# Autodesk Inventor assembly: FinalAssembley
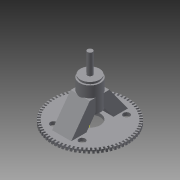
[picture p0: Inventor's stored thumbnail of the model, 180x180]
Saved by Autodesk Inventor 2015 (Build 190159000, 159)
## iProperties
Created: 2015-03-27
Part Number: FinalAssembley
Document SubType Name: Assembly
Designer: WASHHSST
Author: WASHHSST
## Documents named in this file (3)
- E:\DryerGearQuiz\FinalAssembley.iam
- E:\DryerGearQuiz\gear mount.ipt
- E:\DryerGearQuiz\Gear.ipt
## Components (2 placed, 2 different names)
1. gear mount:1 — Mate:1, Mate:2, Mate:3, Mate:4, Mate:5
2. Gear:1 — Mate:1, Mate:2, Mate:3, Mate:4, Mate:5
## Relationships (5: Mate 5)
- Mate:1: gear mount:1 ↔ Gear:1
- Mate:2: gear mount:1 ↔ Gear:1
- Mate:3: gear mount:1 ↔ Gear:1
- Mate:4: gear mount:1 ↔ Gear:1
- Mate:5: gear mount:1 ↔ Gear:1
